# Autodesk Inventor assembly: socket_assembly
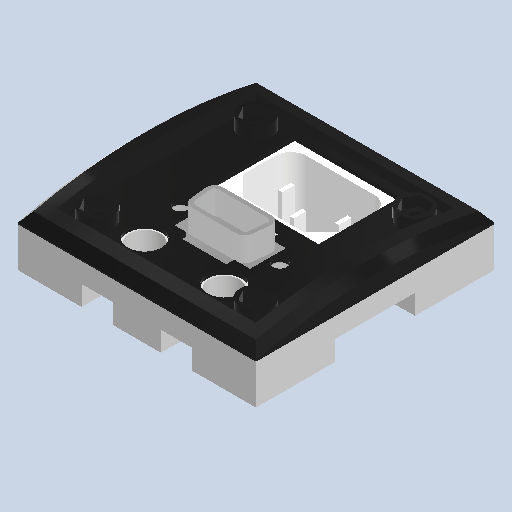
[picture p0: Inventor's stored thumbnail of the model, 512x512]
Saved by Autodesk Inventor 2023 (Build 270158000, 158)
## iProperties
Created: 2023-06-03
Part Number: socket_assembly
Document SubType Name: Assembly
Designer: 310611102
Mass: 50.5678 g
Surface Area: 272.871 cm^2
Volume: 38.8148 cm^3
Density: 1.3028 g/cm^3
Author: 310611102
## Documents named in this file (6)
- C:\Users\310611102\Documents\Inventor\SSR\avionics_2023ver\electronics\socket_assembly.iam
- C:\Users\310611102\Documents\Inventor\SSR\avionics_2023ver\electronics\power_signal_socket.ipt
- C:\Users\310611102\Documents\Inventor\SSR\avionics_2023ver\electronics\Dsub_9pin_female.ipt
- C:\Users\310611102\Documents\Inventor\SSR\avionics_2023ver\electronics\power_socket_24V_2.ipt
- C:\Users\310611102\Documents\Inventor\SSR\avionics_2023ver\electronics\power_signal_socket_cap.ipt
- C:\Users\310611102\Documents\Inventor\SSR\avionics_2023ver\electronics\power_signal_socket_fixed.ipt
## Components (5 placed, 5 different names)
1. power_signal_socket:1 — Insert:5, Mate:1, Mate:2, Mate:3, Insert:6, Mate:4, Mate:5, Mate:6, Insert:7, Insert:8
2. Dsub_9pin_female:1 — Insert:5, Insert:6
3. power_socket_24V_2:1 — Mate:1, Mate:2, Mate:3
4. power_signal_socket_cap:1 — Mate:4, Mate:5, Mate:6
5. power_signal_socket_fixed:1 — Insert:7, Insert:8
## Relationships (10: Mate 6, Insert 4)
- Insert:5: power_signal_socket:1 ↔ Dsub_9pin_female:1
- Mate:1: power_signal_socket:1 ↔ power_socket_24V_2:1
- Mate:2 (0.25 mm): power_signal_socket:1 ↔ power_socket_24V_2:1
- Mate:3 (0.25 mm): power_signal_socket:1 ↔ power_socket_24V_2:1
- Insert:6: power_signal_socket:1 ↔ Dsub_9pin_female:1
- Mate:4: power_signal_socket:1 ↔ power_signal_socket_cap:1
- Mate:5: power_signal_socket:1 ↔ power_signal_socket_cap:1
- Mate:6: power_signal_socket:1 ↔ power_signal_socket_cap:1
- Insert:7: power_signal_socket:1 ↔ power_signal_socket_fixed:1
- Insert:8: power_signal_socket:1 ↔ power_signal_socket_fixed:1
